(part 1 of 2)
# Autodesk Inventor assembly: Main
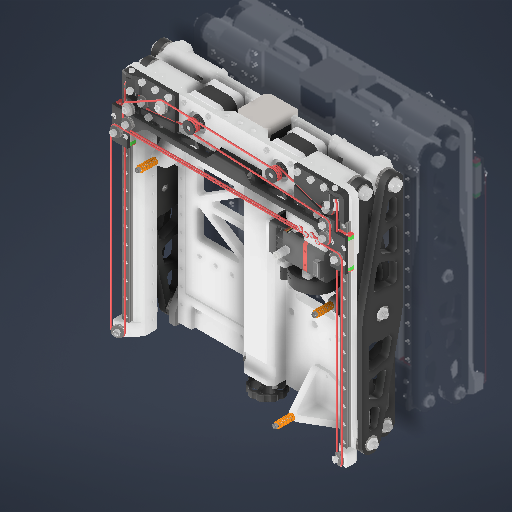
[picture p0: Inventor's stored thumbnail of the model, 512x512]
Saved by Autodesk Inventor 2026.2 (Build 302298000, 298)
## iProperties
Created: 2025-11-20
Part Number: Main
Document SubType Name: Assembly
Designer: gaoet
Author: gaoet
## Documents named in this file (83)
- C:\Users\gaoet\OneDrive\Desktop\Scissor 3D Printer\Main.iam
- C:\Users\gaoet\OneDrive\Desktop\Scissor 3D Printer\Zeee6S22Ah.ipt
- C:\Users\gaoet\Downloads\Positron V3.2.2\42SHD0034-20B\42SHD0034-20B.ipt
- C:\Users\gaoet\OneDrive\Desktop\Scissor 3D Printer\BoundingBox.ipt
- C:\Users\gaoet\OneDrive\Desktop\Scissor 3D Printer\BuildVolume.ipt
- C:\Users\gaoet\OneDrive\Desktop\Scissor 3D Printer\LaptopScaleModel.ipt
- C:\Users\gaoet\OneDrive\Desktop\Scissor 3D Printer\Raspberry PI Zero W\Raspberry PI Zero W.iam
- C:\Users\gaoet\OneDrive\Desktop\Scissor 3D Printer\BTT E3 SKR MINI V3.0\BTT E3 SKR MINI V3.0.iam
- C:\Users\gaoet\OneDrive\Desktop\Scissor 3D Printer\MGN9-H\MGN9-H\MGN9-H.ipt
- C:\Users\gaoet\OneDrive\Desktop\Scissor 3D Printer\ElectronicsBase.ipt
- C:\Users\gaoet\OneDrive\Desktop\Scissor 3D Printer\BottomSlideMount.ipt
- C:\Users\gaoet\OneDrive\Desktop\Scissor 3D Printer\Pololu Stepper with 300mm LeadScrew\Pololu Stepper with 300mm LeadScrew\Pololu Stepper with 300mm LeadScrew.ipt
- C:\Users\gaoet\OneDrive\Desktop\Scissor 3D Printer\nut TR8x8 v7\nut TR8x8 v7\nut TR8x8 v7.ipt
- C:\Users\gaoet\OneDrive\Desktop\Scissor 3D Printer\ZMotorMount.ipt
- C:\Users\gaoet\OneDrive\Desktop\Scissor 3D Printer\BottomSideMountRight.ipt
- C:\Users\gaoet\OneDrive\Desktop\Scissor 3D Printer\ZBridgePlate.ipt
- C:\Users\gaoet\OneDrive\Desktop\Scissor 3D Printer\ScissorArmV2.ipt
- C:\Users\gaoet\OneDrive\Desktop\Scissor 3D Printer\7804K117_Stainless Steel Ball Bearing\7804K117_Stainless Steel Ball Bearing\7804K117_Stainless Steel Ball Bearing.ipt
- C:\Users\gaoet\OneDrive\Desktop\Scissor 3D Printer\92981A207_Alloy Steel Shoulder Screws\92981A207_Alloy Steel Shoulder Screws\92981A207_Alloy Steel Shoulder Screws.ipt
- C:\Users\gaoet\OneDrive\Desktop\Scissor 3D Printer\ShoulderBoltMountV2.ipt
- C:\Users\gaoet\OneDrive\Desktop\Scissor 3D Printer\91415A210_Zinc-Plated Steel Hex Nut\91415A210_Zinc-Plated Steel Hex Nut\91415A210_Zinc-Plated Steel Hex Nut.ipt
- C:\Users\gaoet\OneDrive\Desktop\Scissor 3D Printer\CarriagePivotMount.ipt
- C:\Users\gaoet\OneDrive\Desktop\Scissor 3D Printer\91290A306_Black-Oxide Alloy Steel Socket Head Screw\91290A306_Black-Oxide Alloy Steel Socket Head Screw\91290A306_Black-Oxide Alloy Steel Socket Head Screw.ipt
- C:\Users\gaoet\OneDrive\Desktop\Scissor 3D Printer\PivotWasher.ipt
- C:\Users\gaoet\OneDrive\Desktop\Scissor 3D Printer\90591A255_Zinc-Plated Steel Hex Nut\90591A255_Zinc-Plated Steel Hex Nut\90591A255_Zinc-Plated Steel Hex Nut.ipt
- C:\Users\gaoet\OneDrive\Desktop\Scissor 3D Printer\ScissorArmV2Inner.ipt
- C:\Users\gaoet\OneDrive\Desktop\Scissor 3D Printer\6656K108_Steel Ball Bearing\6656K108_Steel Ball Bearing\6656K108_Steel Ball Bearing.ipt
- C:\Users\gaoet\OneDrive\Desktop\Scissor 3D Printer\91290A168_Black-Oxide Alloy Steel Socket Head Screw\91290A168_Black-Oxide Alloy Steel Socket Head Screw\91290A168_Black-Oxide Alloy Steel Socket Head Screw.ipt
- C:\Users\gaoet\OneDrive\Desktop\Scissor 3D Printer\ThrustBearing.iam
- C:\Users\gaoet\OneDrive\Desktop\Scissor 3D Printer\MGN9-C v2 v0\MGN9-C v2.iam
- C:\Users\gaoet\OneDrive\Desktop\Scissor 3D Printer\UpperCarriagePivotMount.ipt
- C:\Users\gaoet\OneDrive\Desktop\Scissor 3D Printer\MGN9-H\MGN9-H\MGN9-H_MIR.ipt
- C:\Users\gaoet\OneDrive\Desktop\Scissor 3D Printer\91415A210_Zinc-Plated Steel Hex Nut\91415A210_Zinc-Plated Steel Hex Nut\91415A210_Zinc-Plated Steel Hex Nut_MIR.ipt
- C:\Users\gaoet\OneDrive\Desktop\Scissor 3D Printer\7804K117_Stainless Steel Ball Bearing\7804K117_Stainless Steel Ball Bearing\7804K117_Stainless Steel Ball Bearing_MIR.ipt
- C:\Users\gaoet\OneDrive\Desktop\Scissor 3D Printer\ScissorArmV2_MIR.ipt
- C:\Users\gaoet\OneDrive\Desktop\Scissor 3D Printer\92981A207_Alloy Steel Shoulder Screws\92981A207_Alloy Steel Shoulder Screws\92981A207_Alloy Steel Shoulder Screws_MIR.ipt
- C:\Users\gaoet\OneDrive\Desktop\Scissor 3D Printer\CarriagePivotMount_MIR.ipt
- C:\Users\gaoet\OneDrive\Desktop\Scissor 3D Printer\91290A306_Black-Oxide Alloy Steel Socket Head Screw\91290A306_Black-Oxide Alloy Steel Socket Head Screw\91290A306_Black-Oxide Alloy Steel Socket Head Screw_MIR.ipt
- C:\Users\gaoet\OneDrive\Desktop\Scissor 3D Printer\PivotWasher_MIR.ipt
- C:\Users\gaoet\OneDrive\Desktop\Scissor 3D Printer\90591A255_Zinc-Plated Steel Hex Nut\90591A255_Zinc-Plated Steel Hex Nut\90591A255_Zinc-Plated Steel Hex Nut_MIR.ipt
- C:\Users\gaoet\OneDrive\Desktop\Scissor 3D Printer\ScissorArmV2Inner_MIR.ipt
- C:\Users\gaoet\OneDrive\Desktop\Scissor 3D Printer\6656K108_Steel Ball Bearing\6656K108_Steel Ball Bearing\6656K108_Steel Ball Bearing_MIR.ipt
- C:\Users\gaoet\OneDrive\Desktop\Scissor 3D Printer\91290A168_Black-Oxide Alloy Steel Socket Head Screw\91290A168_Black-Oxide Alloy Steel Socket Head Screw\91290A168_Black-Oxide Alloy Steel Socket Head Screw_MIR.ipt
- C:\Users\gaoet\OneDrive\Desktop\Scissor 3D Printer\ThrustBearing_MIR.iam
- C:\Users\gaoet\OneDrive\Desktop\Scissor 3D Printer\MGN9-C v2 v0\MGN9-C v2_MIR.iam
- C:\Users\gaoet\OneDrive\Desktop\Scissor 3D Printer\UpperCarriagePivotMount_MIR.ipt
- C:\Users\gaoet\OneDrive\Desktop\Scissor 3D Printer\91290A110_Black-Oxide Alloy Steel Socket Head Screw\91290A110_Black-Oxide Alloy Steel Socket Head Screw\91290A110_Black-Oxide Alloy Steel Socket Head Screw_MIR.ipt
- C:\Users\gaoet\OneDrive\Desktop\Scissor 3D Printer\GantryRailMount_MIR.ipt
- C:\Users\gaoet\OneDrive\Desktop\Scissor 3D Printer\Extruder.iam
- C:\Users\gaoet\OneDrive\Desktop\Scissor 3D Printer\MGNRail250mm.ipt
- C:\Users\gaoet\OneDrive\Desktop\Scissor 3D Printer\XGantryMount.ipt
- C:\Users\gaoet\OneDrive\Desktop\Scissor 3D Printer\BearingU604.ipt
- C:\Users\gaoet\OneDrive\Desktop\Scissor 3D Printer\90729A168_Passivated 316 Stainless Steel Hex-Drive Flat Head Screw\90729A168_Passivated 316 Stainless Steel Hex-Drive Flat Head Screw\90729A168_Passivated 316 .ipt
- C:\Users\gaoet\OneDrive\Desktop\Scissor 3D Printer\ElevatorPlate.ipt
- C:\Users\gaoet\OneDrive\Desktop\Scissor 3D Printer\ElevatorPlate_MIR.ipt
- C:\Users\gaoet\OneDrive\Desktop\Scissor 3D Printer\XGantryMount_MIR.ipt
- C:\Users\gaoet\OneDrive\Desktop\Scissor 3D Printer\ElevatorShoulderBoltMount.ipt
- C:\Users\gaoet\OneDrive\Desktop\Scissor 3D Printer\ElevatorShoulderBoltMount_MIR.ipt
- C:\Users\gaoet\OneDrive\Desktop\Scissor 3D Printer\Pulley.ipt
- C:\Users\gaoet\OneDrive\Desktop\Scissor 3D Printer\Tensioner.ipt
- C:\Users\gaoet\OneDrive\Desktop\Scissor 3D Printer\PSU.ipt
- C:\Users\gaoet\OneDrive\Desktop\Scissor 3D Printer\LeadScrewArch.ipt
- C:\Users\gaoet\OneDrive\Desktop\Scissor 3D Printer\FrontPanel.ipt
- C:\Users\gaoet\OneDrive\Desktop\Scissor 3D Printer\knob.ipt
- C:\Users\gaoet\OneDrive\Desktop\Scissor 3D Printer\BTT Mini 12864 V1.0\BTT Mini 12864 V1.0\BTT Mini 12864 V1.0.ipt
- C:\Users\gaoet\OneDrive\Desktop\Scissor 3D Printer\BottomSlideMountExtension.ipt
- C:\Users\gaoet\OneDrive\Desktop\Scissor 3D Printer\BottomSlideMountExtension_MIR.ipt
- C:\Users\gaoet\OneDrive\Desktop\Scissor 3D Printer\RightTruss.ipt
- C:\Users\gaoet\OneDrive\Desktop\Scissor 3D Printer\LeftTruss.ipt
- C:\Users\gaoet\OneDrive\Desktop\Scissor 3D Printer\RoutingPlateV2.ipt
- C:\Users\gaoet\OneDrive\Desktop\Scissor 3D Printer\RoutingPlateV2Right.ipt
- C:\Users\gaoet\OneDrive\Desktop\Scissor 3D Printer\ShoulderBoltMountV2_MIR.ipt
- C:\Users\gaoet\OneDrive\Desktop\Scissor 3D Printer\92095A181_NO THREADS_18-8 Stainless Steel Button Head Hex-Drive Screw\92095A181_NO THREADS_18-8 Stainless Steel Button Head Hex-Drive Screw\92095A181_NO THREAD.ipt
- C:\Users\gaoet\OneDrive\Desktop\Scissor 3D Printer\MockCable.ipt
- C:\Users\gaoet\OneDrive\Desktop\Scissor 3D Printer\MockCable2.ipt
- C:\Users\gaoet\OneDrive\Desktop\Scissor 3D Printer\Banana\Banana\Banana.ipt
- C:\Users\gaoet\OneDrive\Desktop\Scissor 3D Printer\GantryRailMount.ipt
- C:\Users\gaoet\OneDrive\Desktop\Scissor 3D Printer\cardboard spool v1\cardboard spool v1\cardboard spool v1.ipt
- C:\Users\gaoet\OneDrive\Desktop\Scissor 3D Printer\LeftLevelBlock.ipt
- C:\Users\gaoet\OneDrive\Desktop\Scissor 3D Printer\RightLevelBlock.ipt
- C:\Users\gaoet\OneDrive\Desktop\Scissor 3D Printer\FrontLevelBlock.ipt
- C:\Users\gaoet\OneDrive\Desktop\Scissor 3D Printer\Spring8x20mm.ipt
- C:\Users\gaoet\OneDrive\Desktop\Polar Plotter\91290A123_Alloy Steel Socket Head Screw\91290A123_Alloy Steel Socket Head Screw.ipt
## Components (336 placed, 82 different names)
1. Zeee6S22Ah:1 — Mate:155, Mate:167
2. 42SHD0034-20B:1 — Mate:132, Flush:39, Mate:143, Mate:148, Flush:46
3. BoundingBox:1 — Mate:41, Flush:14, Mate:42, Angle:2, Mate:149, Flush:47
4. BuildVolume:1
5. LaptopScaleModel:1
6. Raspberry PI Zero W:1 [sub-assembly] — Insert:233, Mate:166, Insert:264, Insert:265
7. BTT E3 SKR MINI V3.0:1 [sub-assembly] — Insert:234, Mate:169
8. MGN9-H:2 — Insert:39, Mate:61, Mate:185
9. MGN9-H:3 — Mate:111, Flush:33, Insert:310
10. MGN9-H:6 — Mate:112, Flush:30, Insert:123, Mate:116
11. ElectronicsBase:1 — Mate:149, Flush:47, Mate:156, Flush:49, Insert:203, Insert:206, Insert:210, Insert:214, Insert:215
12. BottomSlideMount:1 — Mate:13, Mate:20, Insert:10, Insert:11, Mate:139, Mate:140, Flush:43, Insert:207, Insert:208, Insert:213, Mate:167, Mate:170, Mate:171, Flush:50, Insert:261, Insert:328, Flush:53
13. Pololu Stepper with 300mm LeadScrew:1 — Mate:11, Insert:2, Insert:3, Mate:41, Mate:42, Mate:152
14. nut TR8x8 v7:1 — Mate:11, Angle:1
15. ZMotorMount:1 — Insert:2, Insert:3, Mate:13, Mate:20, Mate:22, Insert:10, Insert:11, Mate:23, Mate:24, Angle:1, Mate:72, Mate:82, Mate:154, Insert:266, Insert:267, Insert:268, Insert:269, Insert:270, Insert:271, Insert:272, Insert:303
16. BottomSideMountRight:1 — Mate:22, Mate:23, Mate:24, Flush:14, Mate:52, Mate:53, Mate:54, Angle:8, Mate:138, Mate:141, Mate:153, Mate:168, Mate:169, Mate:172, Insert:283, Flush:52, Insert:329, Flush:54
17. ZBridgePlate:1 — Insert:40, Mate:72, Mate:82, Insert:137, Insert:300, Insert:301, Insert:302
18. 91415A210_Zinc-Plated Steel Hex Nut:1 — Mate:56, Mate:57
19. 7804K117_Stainless Steel Ball Bearing:2 — Mate:70, Insert:52, Insert:325
20. ScissorArmV2:3 — Insert:35, Angle:2, Mate:73, Insert:63, Insert:64, Insert:71, Insert:74, Insert:78, Angle:4
21. 7804K117_Stainless Steel Ball Bearing:3 — Insert:35, Insert:37
22. 92981A207_Alloy Steel Shoulder Screws:3 — Insert:37, Mate:56
23. ShoulderBoltMountV2:1 — Mate:52, Mate:53, Mate:54, Mate:57, Insert:70, Insert:273, Insert:274, Insert:275, Insert:276, Insert:277, Insert:290, Insert:291
24. CarriagePivotMount:1 — Insert:39, Mate:61, Insert:40, Insert:53, Insert:72
25. 91290A306_Black-Oxide Alloy Steel Socket Head Screw:1 — Mate:70, Insert:51
26. PivotWasher:1 — Insert:51, Insert:52
27. 90591A255_Zinc-Plated Steel Hex Nut:1 — Insert:53
28. ScissorArmV2Inner:1 — Mate:73, Insert:68, Mate:74, Insert:73, Angle:4, Insert:316, Insert:325, Insert:326
29. 7804K117_Stainless Steel Ball Bearing:6 — Insert:63, Insert:66
30. 6656K108_Steel Ball Bearing:1 — Insert:64, Insert:65
31. 6656K108_Steel Ball Bearing:2 — Insert:65
32. PivotWasher:3 — Insert:66, Insert:67
33. 91290A168_Black-Oxide Alloy Steel Socket Head Screw:2 — Insert:67
34. 90591A255_Zinc-Plated Steel Hex Nut:2 — Insert:68, Mate:74
35. ThrustBearing:1 [sub-assembly] — Insert:70, Insert:71
36. ThrustBearing:2 [sub-assembly] — Insert:72, Insert:73
37. MGN9-C v2:1 [sub-assembly] — Mate:80, Insert:308, Flush:51
38. 7804K117_Stainless Steel Ball Bearing:7 — Insert:74, Insert:76
39. PivotWasher:4 — Insert:76, Insert:88
40. ThrustBearing:3 [sub-assembly] — Insert:78, Mate:77, Mate:78
41. UpperCarriagePivotMount:1 — Mate:77, Mate:78, Mate:80, Insert:89, Mate:89, Insert:292, Insert:293, Insert:294, Insert:295, Insert:308
42. 91290A306_Black-Oxide Alloy Steel Socket Head Screw:3 — Insert:88
43. 90591A255_Zinc-Plated Steel Hex Nut:3 — Insert:89, Mate:89
44. MGN9-H_MIR:1 — Mate:94, Insert:93
45. 91415A210_Zinc-Plated Steel Hex Nut_MIR:1 — Mate:93
46. 7804K117_Stainless Steel Ball Bearing_MIR:1 — Mate:95, Insert:94, Insert:324
47. ScissorArmV2_MIR:1 — Insert:90, Angle:6, Mate:96, Insert:98, Insert:99, Insert:104, Insert:107, Insert:109
48. 7804K117_Stainless Steel Ball Bearing_MIR:2 — Insert:90, Insert:91
49. 92981A207_Alloy Steel Shoulder Screws_MIR:1 — Mate:93, Insert:91
50. CarriagePivotMount_MIR:1 — Mate:94, Insert:93, Insert:96, Insert:106, Insert:137
51. 91290A306_Black-Oxide Alloy Steel Socket Head Screw_MIR:1 — Mate:95, Insert:95
52. PivotWasher_MIR:1 — Insert:94, Insert:95
53. 90591A255_Zinc-Plated Steel Hex Nut_MIR:1 — Insert:96
54. ScissorArmV2Inner_MIR:1 — Angle:6, Mate:96, Mate:97, Insert:103, Insert:105, Insert:317, Insert:324, Insert:327, Mate:186
55. 7804K117_Stainless Steel Ball Bearing_MIR:3 — Insert:98, Insert:101
56. 6656K108_Steel Ball Bearing_MIR:1 — Insert:99, Insert:100
57. 6656K108_Steel Ball Bearing_MIR:2 — Insert:100, Mate:186
58. PivotWasher_MIR:2 — Insert:101, Insert:102
59. 91290A168_Black-Oxide Alloy Steel Socket Head Screw_MIR:1 — Insert:102
60. 90591A255_Zinc-Plated Steel Hex Nut_MIR:2 — Mate:97, Insert:103
61. ThrustBearing_MIR:1 [sub-assembly] — Insert:104, Insert:241
62. ThrustBearing_MIR:2 [sub-assembly] — Insert:105, Insert:106
63. MGN9-C v2_MIR:1 [sub-assembly] — Mate:99, Mate:122, Flush:35, Insert:307
64. 7804K117_Stainless Steel Ball Bearing_MIR:4 — Insert:107, Insert:108
65. PivotWasher_MIR:3 — Insert:108, Insert:116
66. ThrustBearing_MIR:3 [sub-assembly] — Insert:109, Mate:100, Mate:101
67. UpperCarriagePivotMount_MIR:1 — Mate:99, Mate:100, Mate:101, Mate:106, Insert:117, Insert:296, Insert:297, Insert:298, Insert:299, Insert:307
68. 91290A306_Black-Oxide Alloy Steel Socket Head Screw_MIR:2 — Insert:116
69. 90591A255_Zinc-Plated Steel Hex Nut_MIR:3 — Mate:106, Insert:117
70. Extruder:1 [sub-assembly] — Insert:310, Insert:311, Insert:312, Insert:313, Insert:314
71. MGNRail250mm:3 — Angle:8, Mate:111, Insert:124, Flush:33, Mate:117, Insert:260
72. MGNRail250mm:4 — Mate:112, Flush:30, Insert:152, Mate:128, Insert:319, Insert:320
73. XGantryMount:1 — Insert:123, Mate:116, Insert:124, Mate:117, Insert:138, Insert:139, Insert:140, Insert:141, Mate:126, Insert:142, Insert:145, Mate:131, Flush:42, Insert:183, Insert:184, Mate:174, Angle:12
74. GantryRailMount_MIR:1 — Insert:132, Insert:133, Insert:134, Insert:135, Insert:153
75. MGNRail250mm:6 — Mate:122, Flush:35, Insert:132, Insert:133, Insert:287
76. MGN9-H:7 — Insert:154, Mate:135
77. MGNRail250mm:7 — Insert:134, Insert:135, Insert:247, Mate:188
78. BearingU604:1 — Insert:147, Insert:321
79. BearingU604:2 — Insert:145, Insert:146
80. BearingU604:3 — Mate:126, Insert:142, Insert:143
81. BearingU604:4 — Insert:156, Insert:158, Mate:178
82. BearingU604:5 — Insert:155, Insert:159
83. BearingU604:6 — Insert:153, Insert:157, Mate:179
84. 90729A168_Passivated 316 :1 — Insert:140
85. 90729A168_Passivated 316 :2 — Insert:141
86. 90729A168_Passivated 316 :3 — Insert:139
87. 90729A168_Passivated 316 :4 — Insert:138
88. 91290A306_Black-Oxide Alloy Steel Socket Head Screw:4 — Insert:143, Mate:175
89. 91290A306_Black-Oxide Alloy Steel Socket Head Screw:5 — Insert:146
90. 91290A306_Black-Oxide Alloy Steel Socket Head Screw:6 — Insert:147
91. 90729A168_Passivated 316 :5 — Insert:312
92. 90729A168_Passivated 316 :6 — Insert:313
93. 90729A168_Passivated 316 :7 — Mate:173, Insert:314
94. 90729A168_Passivated 316 :8 — Insert:311
95. ElevatorPlate:1 — Insert:152, Mate:128, Mate:129, Angle:10, Mate:131, Flush:40, Flush:41, Mate:136, Mate:147, Insert:216, Insert:217, Insert:258, Mate:180, Insert:322, Insert:323
96. 42SHD0034-20B:4 — Mate:129, Angle:10, Mate:142, Flush:45, Mate:147
97. ElevatorPlate_MIR:1 — Mate:132, Flush:39, Flush:40, Flush:41, Insert:182, Mate:148, Insert:223, Insert:259, Mate:180, Mate:184, Mate:188
98. XGantryMount_MIR:1 — Insert:154, Mate:135, Flush:42, Insert:155, Insert:156, Insert:160, Insert:161, Insert:162, Insert:163
99. 91290A306_Black-Oxide Alloy Steel Socket Head Screw:7 — Insert:157
100. 91290A306_Black-Oxide Alloy Steel Socket Head Screw:8 — Insert:158
101. 91290A306_Black-Oxide Alloy Steel Socket Head Screw:9 — Insert:159
102. 90729A168_Passivated 316 :9 — Insert:163
103. 90729A168_Passivated 316 :10 — Insert:162
104. 90729A168_Passivated 316 :11 — Insert:161
105. 90729A168_Passivated 316 :12 — Insert:160
106. 92981A207_Alloy Steel Shoulder Screws:4 — Insert:165
107. ThrustBearing:4 [sub-assembly] — Insert:315, Insert:316
108. 7804K117_Stainless Steel Ball Bearing:8 — Insert:165, Insert:326
109. ElevatorShoulderBoltMount:1 — Mate:136, Insert:315, Insert:318
110. 91415A210_Zinc-Plated Steel Hex Nut:3 — Insert:318
111. ElevatorShoulderBoltMount_MIR:1 — Insert:182, Mate:163, Mate:181, Mate:184
112. 92981A207_Alloy Steel Shoulder Screws:5 — Insert:176
113. ThrustBearing:5 [sub-assembly] — Insert:317, Mate:181
114. 7804K117_Stainless Steel Ball Bearing_MIR:5 — Insert:176, Insert:327
115. MGNRail250mm:8 — Mate:138, Mate:141, Mate:185
116. MGNRail250mm:9 — Mate:139, Mate:140, Flush:43, Insert:285
117. BearingU604:10 — Insert:218, Insert:219
118. BearingU604:12 — Insert:187
119. 91290A306_Black-Oxide Alloy Steel Socket Head Screw:20 — Insert:184
120. 91290A306_Black-Oxide Alloy Steel Socket Head Screw:21 — Insert:183
121. Pulley:1 — Mate:142, Flush:45
122. Pulley:2 — Mate:143, Flush:46
123. BearingU604:17 — Insert:229, Insert:231
124. Tensioner:1 — Insert:187, Mate:159, Insert:220, Mate:176, Mate:182
125. PSU:1
126. LeadScrewArch:1 — Mate:152, Mate:153, Mate:154, Insert:194, Mate:155, Insert:263, Insert:306
127. 7804K117_Stainless Steel Ball Bearing:9 — Insert:194
128. knob:1 — Insert:198
129. FrontPanel:2 — Mate:156, Flush:49, Insert:197, Angle:11, Insert:199, Insert:200, Insert:201, Insert:202, Insert:243, Insert:244, Insert:245, Insert:246
130. 7804K117_Stainless Steel Ball Bearing:10 — Insert:197, Insert:198
131. 90729A168_Passivated 316 :13 — Insert:201
132. 90729A168_Passivated 316 :14 — Insert:202
133. BTT Mini 12864 V1.0:1 — Angle:11, Insert:199, Insert:200
134. 90729A168_Passivated 316 :15 — Insert:203
135. 90729A168_Passivated 316 :16 — Insert:206
136. 90729A168_Passivated 316 :17 — Insert:210
137. BottomSlideMountExtension:1 — Insert:207, Insert:208, Insert:212, Insert:233, Mate:166
138. BottomSlideMountExtension_MIR:1 — Insert:211, Insert:234, Mate:168, Mate:172, Insert:284, Insert:330, Mate:187
139. RightTruss:1 — Insert:211, Flush:52
140. LeftTruss:1 — Insert:212, Insert:213
141. 90729A168_Passivated 316 :19 — Insert:214
142. 90729A168_Passivated 316 :20 — Insert:215
143. RoutingPlateV2:1 — Insert:216, Insert:217, Mate:159, Insert:218, Insert:221, Insert:248, Insert:249, Insert:250, Insert:251, Insert:257, Mate:176, Mate:182
144. 91290A306_Black-Oxide Alloy Steel Socket Head Screw:22 — Insert:219
145. 91290A306_Black-Oxide Alloy Steel Socket Head Screw:23 — Insert:220
146. BearingU604:18 — Insert:221, Insert:222
147. 91290A306_Black-Oxide Alloy Steel Socket Head Screw:24 — Insert:222
148. RoutingPlateV2Right:1 — Insert:223, Mate:163, Insert:225, Mate:164, Insert:228, Insert:229, Insert:252, Insert:253, Insert:254, Insert:255, Insert:256, Mate:177, Mate:183
149. BearingU604:19 — Insert:225, Insert:232
150. BearingU604:21
151. Tensioner:2 — Mate:164, Mate:177, Mate:183
152. 91290A306_Black-Oxide Alloy Steel Socket Head Screw:25
153. BearingU604:22 — Insert:228, Insert:230
154. 91290A306_Black-Oxide Alloy Steel Socket Head Screw:26 — Insert:230
155. 91290A306_Black-Oxide Alloy Steel Socket Head Screw:27 — Insert:231
156. 91290A306_Black-Oxide Alloy Steel Socket Head Screw:28 — Insert:232
157. ShoulderBoltMountV2_MIR:1 — Insert:241, Mate:170, Mate:171, Flush:50, Insert:278, Insert:279, Insert:280, Insert:281, Insert:282, Insert:288, Insert:289
158. 90729A168_Passivated 316 :28 — Insert:243
159. 90729A168_Passivated 316 :29 — Insert:244
160. 90729A168_Passivated 316 :30 — Insert:245
161. 90729A168_Passivated 316 :31 — Insert:246
162. 91290A306_Black-Oxide Alloy Steel Socket Head Screw:29 — Insert:249
163. 91290A306_Black-Oxide Alloy Steel Socket Head Screw:30 — Insert:251
164. 91290A306_Black-Oxide Alloy Steel Socket Head Screw:31 — Insert:250
165. 91290A306_Black-Oxide Alloy Steel Socket Head Screw:32 — Insert:248
166. 91290A306_Black-Oxide Alloy Steel Socket Head Screw:33 — Insert:255
167. 91290A306_Black-Oxide Alloy Steel Socket Head Screw:34 — Insert:254
168. 91290A306_Black-Oxide Alloy Steel Socket Head Screw:35 — Insert:252
169. 91290A306_Black-Oxide Alloy Steel Socket Head Screw:36 — Insert:253
170. 91290A110_Black-Oxide Alloy Steel Socket Head Screw_MIR:31 — Insert:257
171. 91290A110_Black-Oxide Alloy Steel Socket Head Screw_MIR:32 — Insert:256
172. 91290A110_Black-Oxide Alloy Steel Socket Head Screw_MIR:60 — Insert:263
173. 91290A110_Black-Oxide Alloy Steel Socket Head Screw_MIR:61 — Insert:264
174. 91290A110_Black-Oxide Alloy Steel Socket Head Screw_MIR:62 — Insert:265
175. 91290A306_Black-Oxide Alloy Steel Socket Head Screw:38 — Insert:266
176. 91290A306_Black-Oxide Alloy Steel Socket Head Screw:39 — Insert:267
177. 91290A306_Black-Oxide Alloy Steel Socket Head Screw:40 — Insert:268
178. 91290A306_Black-Oxide Alloy Steel Socket Head Screw:41 — Insert:269
179. 91290A306_Black-Oxide Alloy Steel Socket Head Screw:42 — Insert:270
180. 91290A306_Black-Oxide Alloy Steel Socket Head Screw:43 — Insert:271
181. 91290A306_Black-Oxide Alloy Steel Socket Head Screw:44 — Insert:272
182. 91290A306_Black-Oxide Alloy Steel Socket Head Screw:46 — Insert:273
183. 91290A306_Black-Oxide Alloy Steel Socket Head Screw:47 — Insert:274
184. 91290A306_Black-Oxide Alloy Steel Socket Head Screw:48 — Insert:275
185. 91290A306_Black-Oxide Alloy Steel Socket Head Screw:49 — Insert:276
186. 91290A306_Black-Oxide Alloy Steel Socket Head Screw:50 — Insert:277
187. 91290A306_Black-Oxide Alloy Steel Socket Head Screw:51 — Insert:278
188. 91290A306_Black-Oxide Alloy Steel Socket Head Screw:52 — Insert:279
189. 91290A306_Black-Oxide Alloy Steel Socket Head Screw:53 — Insert:280
190. 91290A306_Black-Oxide Alloy Steel Socket Head Screw:54 — Insert:281
191. 91290A306_Black-Oxide Alloy Steel Socket Head Screw:55 — Insert:282
192. 91290A306_Black-Oxide Alloy Steel Socket Head Screw:60 — Insert:284
193. 91290A110_Black-Oxide Alloy Steel Socket Head Screw_MIR:115 — Insert:288
194. 91290A110_Black-Oxide Alloy Steel Socket Head Screw_MIR:116 — Insert:289
195. 91290A110_Black-Oxide Alloy Steel Socket Head Screw_MIR:117 — Insert:290
196. 91290A110_Black-Oxide Alloy Steel Socket Head Screw_MIR:118 — Insert:291
197. 92095A181_NO THREAD:1 — Insert:295
198. 92095A181_NO THREAD:2 — Insert:294
199. 92095A181_NO THREAD:3 — Insert:293
200. 92095A181_NO THREAD:4 — Insert:292
201. 92095A181_NO THREAD:5 — Insert:296
202. 92095A181_NO THREAD:6 — Insert:297
203. 92095A181_NO THREAD:7 — Insert:298
204. 92095A181_NO THREAD:8 — Insert:299
205. 91290A110_Black-Oxide Alloy Steel Socket Head Screw_MIR:123
206. 91290A110_Black-Oxide Alloy Steel Socket Head Screw_MIR:124
207. MockCable:1 — Mate:173, Mate:174, Angle:12, Mate:175
208. MockCable2:1 — Mate:178, Mate:179
209. Banana:1
210. GantryRailMount:1 — Insert:319, Insert:320, Insert:321
211. MGNRail250mm:10 — Insert:322, Insert:323, Flush:51
212. cardboard spool v1:1
213. LeftLevelBlock:1 — Insert:328, Flush:53, Insert:333
214. RightLevelBlock:1 — Insert:329, Flush:54, Insert:332
215. FrontLevelBlock:1 — Insert:330, Mate:187, Insert:331
216. Spring8x20mm:1 — Insert:331, Insert:334
217. Spring8x20mm:2 — Insert:333, Insert:335
218. Spring8x20mm:3 — Insert:332, Insert:336
219. Pololu Stepper with 300mm LeadScrew:2
220. 91290A123_Alloy Steel Socket Head Screw:1 — Insert:335
221. 91290A123_Alloy Steel Socket Head Screw:2 — Insert:336
222. 91290A123_Alloy Steel Socket Head Screw:3 — Insert:334
223. 91290A110_Black-Oxide Alloy Steel Socket Head Screw_MIR:5 — Insert:247
224. 91290A110_Black-Oxide Alloy Steel Socket Head Screw_MIR:18
225. 91290A110_Black-Oxide Alloy Steel Socket Head Screw_MIR:6
226. 91290A110_Black-Oxide Alloy Steel Socket Head Screw_MIR:19
227. 91290A110_Black-Oxide Alloy Steel Socket Head Screw_MIR:7
228. 91290A110_Black-Oxide Alloy Steel Socket Head Screw_MIR:20
229. 91290A110_Black-Oxide Alloy Steel Socket Head Screw_MIR:8
230. 91290A110_Black-Oxide Alloy Steel Socket Head Screw_MIR:21
231. 91290A110_Black-Oxide Alloy Steel Socket Head Screw_MIR:9
232. 91290A110_Black-Oxide Alloy Steel Socket Head Screw_MIR:22
233. 91290A110_Black-Oxide Alloy Steel Socket Head Screw_MIR:10
234. 91290A110_Black-Oxide Alloy Steel Socket Head Screw_MIR:23
235. 91290A110_Black-Oxide Alloy Steel Socket Head Screw_MIR:11
236. 91290A110_Black-Oxide Alloy Steel Socket Head Screw_MIR:24
237. 91290A110_Black-Oxide Alloy Steel Socket Head Screw_MIR:12
238. 91290A110_Black-Oxide Alloy Steel Socket Head Screw_MIR:25
239. 91290A110_Black-Oxide Alloy Steel Socket Head Screw_MIR:13
240. 91290A110_Black-Oxide Alloy Steel Socket Head Screw_MIR:26
241. 91290A110_Black-Oxide Alloy Steel Socket Head Screw_MIR:14
242. 91290A110_Black-Oxide Alloy Steel Socket Head Screw_MIR:27
243. 91290A110_Black-Oxide Alloy Steel Socket Head Screw_MIR:15
244. 91290A110_Black-Oxide Alloy Steel Socket Head Screw_MIR:28
245. 91290A110_Black-Oxide Alloy Steel Socket Head Screw_MIR:16
246. 91290A110_Black-Oxide Alloy Steel Socket Head Screw_MIR:29
247. 91290A110_Black-Oxide Alloy Steel Socket Head Screw_MIR:17
248. 91290A110_Black-Oxide Alloy Steel Socket Head Screw_MIR:30
249. 91290A110_Black-Oxide Alloy Steel Socket Head Screw_MIR:41 — Insert:260
250. 91290A110_Black-Oxide Alloy Steel Socket Head Screw_MIR:42
251. 91290A110_Black-Oxide Alloy Steel Socket Head Screw_MIR:43
252. 91290A110_Black-Oxide Alloy Steel Socket Head Screw_MIR:44
253. 91290A110_Black-Oxide Alloy Steel Socket Head Screw_MIR:45
254. 91290A110_Black-Oxide Alloy Steel Socket Head Screw_MIR:46
255. 91290A110_Black-Oxide Alloy Steel Socket Head Screw_MIR:47
256. 91290A110_Black-Oxide Alloy Steel Socket Head Screw_MIR:48
257. 91290A110_Black-Oxide Alloy Steel Socket Head Screw_MIR:49
258. 91290A110_Black-Oxide Alloy Steel Socket Head Screw_MIR:50
259. 91290A110_Black-Oxide Alloy Steel Socket Head Screw_MIR:51
260. 91290A110_Black-Oxide Alloy Steel Socket Head Screw_MIR:52
261. 91290A110_Black-Oxide Alloy Steel Socket Head Screw_MIR:53
262. 91290A110_Black-Oxide Alloy Steel Socket Head Screw_MIR:54 — Insert:261
263. 91290A110_Black-Oxide Alloy Steel Socket Head Screw_MIR:55
264. 91290A110_Black-Oxide Alloy Steel Socket Head Screw_MIR:56
265. 91290A306_Black-Oxide Alloy Steel Socket Head Screw:56 — Insert:283
266. 91290A306_Black-Oxide Alloy Steel Socket Head Screw:57
267. 91290A306_Black-Oxide Alloy Steel Socket Head Screw:58
268. 91290A306_Black-Oxide Alloy Steel Socket Head Screw:59
269. 91290A110_Black-Oxide Alloy Steel Socket Head Screw_MIR:63 — Insert:285
270. 91290A110_Black-Oxide Alloy Steel Socket Head Screw_MIR:64
271. 91290A110_Black-Oxide Alloy Steel Socket Head Screw_MIR:65
272. 91290A110_Black-Oxide Alloy Steel Socket Head Screw_MIR:66
273. 91290A110_Black-Oxide Alloy Steel Socket Head Screw_MIR:67
274. 91290A110_Black-Oxide Alloy Steel Socket Head Screw_MIR:68
275. 91290A110_Black-Oxide Alloy Steel Socket Head Screw_MIR:69
276. 91290A110_Black-Oxide Alloy Steel Socket Head Screw_MIR:70
277. 91290A110_Black-Oxide Alloy Steel Socket Head Screw_MIR:71
278. 91290A110_Black-Oxide Alloy Steel Socket Head Screw_MIR:72
279. 91290A110_Black-Oxide Alloy Steel Socket Head Screw_MIR:73
280. 91290A110_Black-Oxide Alloy Steel Socket Head Screw_MIR:74
281. 91290A110_Black-Oxide Alloy Steel Socket Head Screw_MIR:75
282. 91290A110_Black-Oxide Alloy Steel Socket Head Screw_MIR:76
283. 91290A110_Black-Oxide Alloy Steel Socket Head Screw_MIR:77
284. 91290A110_Black-Oxide Alloy Steel Socket Head Screw_MIR:78
285. 91290A110_Black-Oxide Alloy Steel Socket Head Screw_MIR:79
286. 91290A110_Black-Oxide Alloy Steel Socket Head Screw_MIR:80
287. 91290A110_Black-Oxide Alloy Steel Socket Head Screw_MIR:81
288. 91290A110_Black-Oxide Alloy Steel Socket Head Screw_MIR:82
289. 91290A110_Black-Oxide Alloy Steel Socket Head Screw_MIR:83
290. 91290A110_Black-Oxide Alloy Steel Socket Head Screw_MIR:84
291. 91290A110_Black-Oxide Alloy Steel Socket Head Screw_MIR:85
292. 91290A110_Black-Oxide Alloy Steel Socket Head Screw_MIR:86
293. 91290A110_Black-Oxide Alloy Steel Socket Head Screw_MIR:87
294. 91290A110_Black-Oxide Alloy Steel Socket Head Screw_MIR:88
295. 91290A110_Black-Oxide Alloy Steel Socket Head Screw_MIR:102 — Insert:287
296. 91290A110_Black-Oxide Alloy Steel Socket Head Screw_MIR:103
297. 91290A110_Black-Oxide Alloy Steel Socket Head Screw_MIR:104
298. 91290A110_Black-Oxide Alloy Steel Socket Head Screw_MIR:105
299. 91290A110_Black-Oxide Alloy Steel Socket Head Screw_MIR:106
300. 91290A110_Black-Oxide Alloy Steel Socket Head Screw_MIR:107
301. 91290A110_Black-Oxide Alloy Steel Socket Head Screw_MIR:108
302. 91290A110_Black-Oxide Alloy Steel Socket Head Screw_MIR:109
303. 91290A110_Black-Oxide Alloy Steel Socket Head Screw_MIR:110
304. 91290A110_Black-Oxide Alloy Steel Socket Head Screw_MIR:111
305. 91290A110_Black-Oxide Alloy Steel Socket Head Screw_MIR:112
306. 91290A110_Black-Oxide Alloy Steel Socket Head Screw_MIR:113
307. 91290A110_Black-Oxide Alloy Steel Socket Head Screw_MIR:114
308. 92095A181_NO THREAD:9 — Insert:300
309. 92095A181_NO THREAD:12
310. 92095A181_NO THREAD:13
311. 92095A181_NO THREAD:14
312. 92095A181_NO THREAD:10 — Insert:302
313. 92095A181_NO THREAD:15
314. 92095A181_NO THREAD:16
315. 92095A181_NO THREAD:17
316. 92095A181_NO THREAD:11 — Insert:301
317. 92095A181_NO THREAD:18
318. 92095A181_NO THREAD:19
319. 92095A181_NO THREAD:20
320. 91290A110_Black-Oxide Alloy Steel Socket Head Screw_MIR:119 — Insert:303
321. 91290A110_Black-Oxide Alloy Steel Socket Head Screw_MIR:120
322. 91290A110_Black-Oxide Alloy Steel Socket Head Screw_MIR:121
323. 91290A110_Black-Oxide Alloy Steel Socket Head Screw_MIR:122
324. 91290A110_Black-Oxide Alloy Steel Socket Head Screw_MIR:125 — Insert:306
325. 91290A110_Black-Oxide Alloy Steel Socket Head Screw_MIR:126
326. 91290A110_Black-Oxide Alloy Steel Socket Head Screw_MIR:127
327. 91290A110_Black-Oxide Alloy Steel Socket Head Screw_MIR:128
328. 91290A110_Black-Oxide Alloy Steel Socket Head Screw_MIR:129
329. 91290A110_Black-Oxide Alloy Steel Socket Head Screw_MIR:33 — Insert:258
330. 91290A110_Black-Oxide Alloy Steel Socket Head Screw_MIR:130
331. 91290A110_Black-Oxide Alloy Steel Socket Head Screw_MIR:131
332. 91290A110_Black-Oxide Alloy Steel Socket Head Screw_MIR:132
333. 91290A110_Black-Oxide Alloy Steel Socket Head Screw_MIR:37 — Insert:259
334. 91290A110_Black-Oxide Alloy Steel Socket Head Screw_MIR:133
335. 91290A110_Black-Oxide Alloy Steel Socket Head Screw_MIR:134
336. 91290A110_Black-Oxide Alloy Steel Socket Head Screw_MIR:135
## Component patterns: (26 elements, first: 91290A110_Black-Oxide Alloy Steel Socket Head Screw_MIR:5), (13 elements, first: 91290A110_Black-Oxide Alloy Steel Socket Head Screw_MIR:41), (3 elements, first: 91290A110_Black-Oxide Alloy Steel Socket Head Screw_MIR:54), (4 elements, first: 91290A306_Black-Oxide Alloy Steel Socket Head Screw:56), (26 elements, first: 91290A110_Black-Oxide Alloy Steel Socket Head Screw_MIR:63), (13 elements, first: 91290A110_Black-Oxide Alloy Steel Socket Head Screw_MIR:102), (4 elements, first: 92095A181_NO THREAD:9), (4 elements, first: 92095A181_NO THREAD:10), (4 elements, first: 92095A181_NO THREAD:11), (4 elements, first: 91290A110_Black-Oxide Alloy Steel Socket Head Screw_MIR:119), (5 elements, first: 91290A110_Black-Oxide Alloy Steel Socket Head Screw_MIR:125), (4 elements, first: 91290A110_Black-Oxide Alloy Steel Socket Head Screw_MIR:33), (4 elements, first: 91290A110_Black-Oxide Alloy Steel Socket Head Screw_MIR:37)
## Relationships (317: Insert 205, Mate 85, Flush 19, Angle 8)
- Mate:11: Pololu Stepper with 300mm LeadScrew:1 ↔ nut TR8x8 v7:1
- Insert:2: Pololu Stepper with 300mm LeadScrew:1 ↔ ZMotorMount:1
- Insert:3: Pololu Stepper with 300mm LeadScrew:1 ↔ ZMotorMount:1
- Mate:13: BottomSlideMount:1 ↔ ZMotorMount:1
- Mate:20: BottomSlideMount:1 ↔ ZMotorMount:1
- Mate:22: ZMotorMount:1 ↔ BottomSideMountRight:1
- Insert:10: BottomSlideMount:1 ↔ ZMotorMount:1
- Insert:11: BottomSlideMount:1 ↔ ZMotorMount:1
- Mate:23: ZMotorMount:1 ↔ BottomSideMountRight:1
- Mate:24: ZMotorMount:1 ↔ BottomSideMountRight:1
- Angle:1 (0 deg): nut TR8x8 v7:1 ↔ ZMotorMount:1
- Mate:41: BoundingBox:1 ↔ Pololu Stepper with 300mm LeadScrew:1
- Flush:14 (14 mm): BoundingBox:1 ↔ BottomSideMountRight:1
- Mate:42: BoundingBox:1 ↔ Pololu Stepper with 300mm LeadScrew:1
- Insert:35: ScissorArmV2:3 ↔ 7804K117_Stainless Steel Ball Bearing:3
- Insert:37: 7804K117_Stainless Steel Ball Bearing:3 ↔ 92981A207_Alloy Steel Shoulder Screws:3
- Mate:52: BottomSideMountRight:1 ↔ ShoulderBoltMountV2:1
- Mate:53: BottomSideMountRight:1 ↔ ShoulderBoltMountV2:1
- Mate:54: BottomSideMountRight:1 ↔ ShoulderBoltMountV2:1
- Mate:56: 91415A210_Zinc-Plated Steel Hex Nut:1 ↔ 92981A207_Alloy Steel Shoulder Screws:3
- Mate:57: 91415A210_Zinc-Plated Steel Hex Nut:1 ↔ ShoulderBoltMountV2:1
- Angle:2 (186 deg): BoundingBox:1 ↔ ScissorArmV2:3
- Insert:39: MGN9-H:2 ↔ CarriagePivotMount:1
- Mate:61: MGN9-H:2 ↔ CarriagePivotMount:1
- Insert:40: ZBridgePlate:1 ↔ CarriagePivotMount:1
- Mate:70: 7804K117_Stainless Steel Ball Bearing:2 ↔ 91290A306_Black-Oxide Alloy Steel Socket Head Screw:1
- Insert:51: 91290A306_Black-Oxide Alloy Steel Socket Head Screw:1 ↔ PivotWasher:1
- Insert:52: 7804K117_Stainless Steel Ball Bearing:2 ↔ PivotWasher:1
- Insert:53: CarriagePivotMount:1 ↔ 90591A255_Zinc-Plated Steel Hex Nut:1
- Mate:72: ZMotorMount:1 ↔ ZBridgePlate:1
- Mate:73: ScissorArmV2:3 ↔ ScissorArmV2Inner:1
- Insert:63: ScissorArmV2:3 ↔ 7804K117_Stainless Steel Ball Bearing:6
- Insert:64: ScissorArmV2:3 ↔ 6656K108_Steel Ball Bearing:1
- Insert:65: 6656K108_Steel Ball Bearing:1 ↔ 6656K108_Steel Ball Bearing:2
- Insert:66: 7804K117_Stainless Steel Ball Bearing:6 ↔ PivotWasher:3
- Insert:67: PivotWasher:3 ↔ 91290A168_Black-Oxide Alloy Steel Socket Head Screw:2
- Insert:68: ScissorArmV2Inner:1 ↔ 90591A255_Zinc-Plated Steel Hex Nut:2
- Mate:74: ScissorArmV2Inner:1 ↔ 90591A255_Zinc-Plated Steel Hex Nut:2
- Insert:70: ShoulderBoltMountV2:1 ↔ ThrustBearing:1
- Insert:71: ScissorArmV2:3 ↔ ThrustBearing:1
- Insert:72: CarriagePivotMount:1 ↔ ThrustBearing:2
- Insert:73: ScissorArmV2Inner:1 ↔ ThrustBearing:2
- Insert:74: ScissorArmV2:3 ↔ 7804K117_Stainless Steel Ball Bearing:7
- Insert:76: 7804K117_Stainless Steel Ball Bearing:7 ↔ PivotWasher:4
- Insert:78: ScissorArmV2:3 ↔ ThrustBearing:3
- Mate:77: ThrustBearing:3 ↔ UpperCarriagePivotMount:1
- Mate:78: ThrustBearing:3 ↔ UpperCarriagePivotMount:1
- Angle:4 (0 deg): ScissorArmV2:3 ↔ ScissorArmV2Inner:1
- Mate:80: MGN9-C v2:1 ↔ UpperCarriagePivotMount:1
- Mate:82 (178.4935 mm): ZMotorMount:1 ↔ ZBridgePlate:1
- Insert:88: PivotWasher:4 ↔ 91290A306_Black-Oxide Alloy Steel Socket Head Screw:3
- Insert:89: UpperCarriagePivotMount:1 ↔ 90591A255_Zinc-Plated Steel Hex Nut:3
- Mate:89: UpperCarriagePivotMount:1 ↔ 90591A255_Zinc-Plated Steel Hex Nut:3
- Insert:90: ScissorArmV2_MIR:1 ↔ 7804K117_Stainless Steel Ball Bearing_MIR:2
- Mate:93: 91415A210_Zinc-Plated Steel Hex Nut_MIR:1 ↔ 92981A207_Alloy Steel Shoulder Screws_MIR:1
- Insert:91: 7804K117_Stainless Steel Ball Bearing_MIR:2 ↔ 92981A207_Alloy Steel Shoulder Screws_MIR:1
- Mate:94: MGN9-H_MIR:1 ↔ CarriagePivotMount_MIR:1
- Insert:93: MGN9-H_MIR:1 ↔ CarriagePivotMount_MIR:1
- Mate:95: 7804K117_Stainless Steel Ball Bearing_MIR:1 ↔ 91290A306_Black-Oxide Alloy Steel Socket Head Screw_MIR:1
- Insert:94: 7804K117_Stainless Steel Ball Bearing_MIR:1 ↔ PivotWasher_MIR:1
- Insert:95: 91290A306_Black-Oxide Alloy Steel Socket Head Screw_MIR:1 ↔ PivotWasher_MIR:1
- Insert:96: CarriagePivotMount_MIR:1 ↔ 90591A255_Zinc-Plated Steel Hex Nut_MIR:1
- Angle:6 (0 deg): ScissorArmV2_MIR:1 ↔ ScissorArmV2Inner_MIR:1
- Mate:96: ScissorArmV2_MIR:1 ↔ ScissorArmV2Inner_MIR:1
- Insert:98: ScissorArmV2_MIR:1 ↔ 7804K117_Stainless Steel Ball Bearing_MIR:3
- Insert:99: ScissorArmV2_MIR:1 ↔ 6656K108_Steel Ball Bearing_MIR:1
- Insert:100: 6656K108_Steel Ball Bearing_MIR:1 ↔ 6656K108_Steel Ball Bearing_MIR:2
- Insert:101: 7804K117_Stainless Steel Ball Bearing_MIR:3 ↔ PivotWasher_MIR:2
- Insert:102: PivotWasher_MIR:2 ↔ 91290A168_Black-Oxide Alloy Steel Socket Head Screw_MIR:1
- Mate:97: ScissorArmV2Inner_MIR:1 ↔ 90591A255_Zinc-Plated Steel Hex Nut_MIR:2
- Insert:103: ScissorArmV2Inner_MIR:1 ↔ 90591A255_Zinc-Plated Steel Hex Nut_MIR:2
- Insert:104: ScissorArmV2_MIR:1 ↔ ThrustBearing_MIR:1
- Insert:105: ScissorArmV2Inner_MIR:1 ↔ ThrustBearing_MIR:2
- Insert:106: CarriagePivotMount_MIR:1 ↔ ThrustBearing_MIR:2
- Insert:107: ScissorArmV2_MIR:1 ↔ 7804K117_Stainless Steel Ball Bearing_MIR:4
- Insert:108: 7804K117_Stainless Steel Ball Bearing_MIR:4 ↔ PivotWasher_MIR:3
- Insert:109: ScissorArmV2_MIR:1 ↔ ThrustBearing_MIR:3
- Mate:99: MGN9-C v2_MIR:1 ↔ UpperCarriagePivotMount_MIR:1
- Mate:100: ThrustBearing_MIR:3 ↔ UpperCarriagePivotMount_MIR:1
- Mate:101: ThrustBearing_MIR:3 ↔ UpperCarriagePivotMount_MIR:1
- Insert:116: PivotWasher_MIR:3 ↔ 91290A306_Black-Oxide Alloy Steel Socket Head Screw_MIR:2
- Mate:106: UpperCarriagePivotMount_MIR:1 ↔ 90591A255_Zinc-Plated Steel Hex Nut_MIR:3
- Insert:117: UpperCarriagePivotMount_MIR:1 ↔ 90591A255_Zinc-Plated Steel Hex Nut_MIR:3
- Angle:8 (0 deg): BottomSideMountRight:1 ↔ MGNRail250mm:3
- Mate:111: MGN9-H:3 ↔ MGNRail250mm:3
- Mate:112: MGN9-H:6 ↔ MGNRail250mm:4
- Flush:30 (5.5 mm): MGN9-H:6 ↔ MGNRail250mm:4
- Insert:123: MGN9-H:6 ↔ XGantryMount:1
- Mate:116: MGN9-H:6 ↔ XGantryMount:1
- Insert:124: MGNRail250mm:3 ↔ XGantryMount:1
- Flush:33 (-5.5 mm): MGN9-H:3 ↔ MGNRail250mm:3
- Mate:117: MGNRail250mm:3 ↔ XGantryMount:1
- Mate:122: MGN9-C v2_MIR:1 ↔ MGNRail250mm:6
- Flush:35 (5.5 mm): MGN9-C v2_MIR:1 ↔ MGNRail250mm:6
- Insert:132: GantryRailMount_MIR:1 ↔ MGNRail250mm:6
- Insert:133: GantryRailMount_MIR:1 ↔ MGNRail250mm:6
- [Mate]: MGN9-H:7 ↔ MGNRail250mm:7
- [Flush] (5.5 mm): MGN9-H:7 ↔ MGNRail250mm:7
- Insert:134: GantryRailMount_MIR:1 ↔ MGNRail250mm:7
- Insert:135: GantryRailMount_MIR:1 ↔ MGNRail250mm:7
- Insert:137: ZBridgePlate:1 ↔ CarriagePivotMount_MIR:1
- Insert:138: XGantryMount:1 ↔ 90729A168_Passivated 316 :4
- Insert:139: XGantryMount:1 ↔ 90729A168_Passivated 316 :3
- Insert:140: XGantryMount:1 ↔ 90729A168_Passivated 316 :1
- Insert:141: XGantryMount:1 ↔ 90729A168_Passivated 316 :2
- Mate:126: XGantryMount:1 ↔ BearingU604:3
- Insert:142: XGantryMount:1 ↔ BearingU604:3
- Insert:143: BearingU604:3 ↔ 91290A306_Black-Oxide Alloy Steel Socket Head Screw:4
- Insert:145: XGantryMount:1 ↔ BearingU604:2
- Insert:146: BearingU604:2 ↔ 91290A306_Black-Oxide Alloy Steel Socket Head Screw:5
- Insert:147: BearingU604:1 ↔ 91290A306_Black-Oxide Alloy Steel Socket Head Screw:6
- Insert:152: MGNRail250mm:4 ↔ ElevatorPlate:1
- Mate:128: MGNRail250mm:4 ↔ ElevatorPlate:1
- Mate:129: ElevatorPlate:1 ↔ 42SHD0034-20B:4
- Angle:10 (0 deg): ElevatorPlate:1 ↔ 42SHD0034-20B:4
- Mate:131: XGantryMount:1 ↔ ElevatorPlate:1
- Mate:132: 42SHD0034-20B:1 ↔ ElevatorPlate_MIR:1
- Flush:39: 42SHD0034-20B:1 ↔ ElevatorPlate_MIR:1
- Flush:40: ElevatorPlate:1 ↔ ElevatorPlate_MIR:1
- Flush:41: ElevatorPlate:1 ↔ ElevatorPlate_MIR:1
- Insert:153: GantryRailMount_MIR:1 ↔ BearingU604:6
- Insert:154: MGN9-H:7 ↔ XGantryMount_MIR:1
- Mate:135: MGN9-H:7 ↔ XGantryMount_MIR:1
- Flush:42: XGantryMount:1 ↔ XGantryMount_MIR:1
- Insert:155: BearingU604:5 ↔ XGantryMount_MIR:1
- Insert:156: BearingU604:4 ↔ XGantryMount_MIR:1
- Insert:157: BearingU604:6 ↔ 91290A306_Black-Oxide Alloy Steel Socket Head Screw:7
- Insert:158: BearingU604:4 ↔ 91290A306_Black-Oxide Alloy Steel Socket Head Screw:8
- Insert:159: BearingU604:5 ↔ 91290A306_Black-Oxide Alloy Steel Socket Head Screw:9
- Insert:160: XGantryMount_MIR:1 ↔ 90729A168_Passivated 316 :12
- Insert:161: XGantryMount_MIR:1 ↔ 90729A168_Passivated 316 :11
- Insert:162: XGantryMount_MIR:1 ↔ 90729A168_Passivated 316 :10
- Insert:163: XGantryMount_MIR:1 ↔ 90729A168_Passivated 316 :9
- Insert:165: 92981A207_Alloy Steel Shoulder Screws:4 ↔ 7804K117_Stainless Steel Ball Bearing:8
- Mate:136: ElevatorPlate:1 ↔ ElevatorShoulderBoltMount:1
- Insert:176: 92981A207_Alloy Steel Shoulder Screws:5 ↔ 7804K117_Stainless Steel Ball Bearing_MIR:5
- Insert:182: ElevatorPlate_MIR:1 ↔ ElevatorShoulderBoltMount_MIR:1
- Mate:138: BottomSideMountRight:1 ↔ MGNRail250mm:8
- Mate:139: BottomSlideMount:1 ↔ MGNRail250mm:9
- Mate:140: BottomSlideMount:1 ↔ MGNRail250mm:9
- Flush:43: BottomSlideMount:1 ↔ MGNRail250mm:9
- Mate:141: BottomSideMountRight:1 ↔ MGNRail250mm:8
- Insert:183: XGantryMount:1 ↔ 91290A306_Black-Oxide Alloy Steel Socket Head Screw:21
- Insert:184: XGantryMount:1 ↔ 91290A306_Black-Oxide Alloy Steel Socket Head Screw:20
- Mate:142: 42SHD0034-20B:4 ↔ Pulley:1
- Mate:143: 42SHD0034-20B:1 ↔ Pulley:2
- Insert:187: BearingU604:12 ↔ Tensioner:1
- Flush:45: 42SHD0034-20B:4 ↔ Pulley:1
- Mate:147: ElevatorPlate:1 ↔ 42SHD0034-20B:4
- Mate:148: 42SHD0034-20B:1 ↔ ElevatorPlate_MIR:1
- Flush:46: 42SHD0034-20B:1 ↔ Pulley:2
- Mate:149: BoundingBox:1 ↔ ElectronicsBase:1
- Mate:152: Pololu Stepper with 300mm LeadScrew:1 ↔ LeadScrewArch:1
- Mate:153: BottomSideMountRight:1 ↔ LeadScrewArch:1
- Mate:154: ZMotorMount:1 ↔ LeadScrewArch:1
- Insert:194: LeadScrewArch:1 ↔ 7804K117_Stainless Steel Ball Bearing:9
- Mate:155: Zeee6S22Ah:1 ↔ LeadScrewArch:1
- Flush:47: BoundingBox:1 ↔ ElectronicsBase:1
- Mate:156: ElectronicsBase:1 ↔ FrontPanel:2
- Flush:49: ElectronicsBase:1 ↔ FrontPanel:2
- Insert:197: FrontPanel:2 ↔ 7804K117_Stainless Steel Ball Bearing:10
- Insert:198: knob:1 ↔ 7804K117_Stainless Steel Ball Bearing:10
- Angle:11 (0 deg): FrontPanel:2 ↔ BTT Mini 12864 V1.0:1
- Insert:199: FrontPanel:2 ↔ BTT Mini 12864 V1.0:1
- Insert:200: FrontPanel:2 ↔ BTT Mini 12864 V1.0:1
- Insert:201: FrontPanel:2 ↔ 90729A168_Passivated 316 :13
- Insert:202: FrontPanel:2 ↔ 90729A168_Passivated 316 :14
- Insert:203: ElectronicsBase:1 ↔ 90729A168_Passivated 316 :15
- Insert:206: ElectronicsBase:1 ↔ 90729A168_Passivated 316 :16
- Insert:207: BottomSlideMount:1 ↔ BottomSlideMountExtension:1
- Insert:208: BottomSlideMount:1 ↔ BottomSlideMountExtension:1
- Insert:210: ElectronicsBase:1 ↔ 90729A168_Passivated 316 :17
- Insert:211: BottomSlideMountExtension_MIR:1 ↔ RightTruss:1
- Insert:212: BottomSlideMountExtension:1 ↔ LeftTruss:1
- Insert:213: BottomSlideMount:1 ↔ LeftTruss:1
- Insert:214: ElectronicsBase:1 ↔ 90729A168_Passivated 316 :19
- Insert:215: ElectronicsBase:1 ↔ 90729A168_Passivated 316 :20
- Insert:216: ElevatorPlate:1 ↔ RoutingPlateV2:1
- Insert:217: ElevatorPlate:1 ↔ RoutingPlateV2:1
- Mate:159 (0.1 mm): Tensioner:1 ↔ RoutingPlateV2:1
- Insert:218: BearingU604:10 ↔ RoutingPlateV2:1
- Insert:219: BearingU604:10 ↔ 91290A306_Black-Oxide Alloy Steel Socket Head Screw:22
- Insert:220: Tensioner:1 ↔ 91290A306_Black-Oxide Alloy Steel Socket Head Screw:23
- Insert:221: RoutingPlateV2:1 ↔ BearingU604:18
- Insert:222: BearingU604:18 ↔ 91290A306_Black-Oxide Alloy Steel Socket Head Screw:24
- Insert:223: ElevatorPlate_MIR:1 ↔ RoutingPlateV2Right:1
- Mate:163: ElevatorShoulderBoltMount_MIR:1 ↔ RoutingPlateV2Right:1
- Insert:225: RoutingPlateV2Right:1 ↔ BearingU604:19
- [Insert]: BearingU604:21 ↔ Tensioner:2
- [Insert]: Tensioner:2 ↔ 91290A306_Black-Oxide Alloy Steel Socket Head Screw:25
- Mate:164 (0.1 mm): RoutingPlateV2Right:1 ↔ Tensioner:2
- Insert:228: RoutingPlateV2Right:1 ↔ BearingU604:22
- Insert:229: BearingU604:17 ↔ RoutingPlateV2Right:1
- Insert:230: BearingU604:22 ↔ 91290A306_Black-Oxide Alloy Steel Socket Head Screw:26
- Insert:231: BearingU604:17 ↔ 91290A306_Black-Oxide Alloy Steel Socket Head Screw:27
- Insert:232: BearingU604:19 ↔ 91290A306_Black-Oxide Alloy Steel Socket Head Screw:28
- Insert:233: Raspberry PI Zero W:1 ↔ BottomSlideMountExtension:1
- Mate:166: Raspberry PI Zero W:1 ↔ BottomSlideMountExtension:1
- Mate:167: Zeee6S22Ah:1 ↔ BottomSlideMount:1
- Insert:234 (3 mm): BTT E3 SKR MINI V3.0:1 ↔ BottomSlideMountExtension_MIR:1
- Mate:168: BottomSideMountRight:1 ↔ BottomSlideMountExtension_MIR:1
- Mate:169: BTT E3 SKR MINI V3.0:1 ↔ BottomSideMountRight:1
- Insert:241: ThrustBearing_MIR:1 ↔ ShoulderBoltMountV2_MIR:1
- Mate:170: BottomSlideMount:1 ↔ ShoulderBoltMountV2_MIR:1
- Mate:171: BottomSlideMount:1 ↔ ShoulderBoltMountV2_MIR:1
- Flush:50: BottomSlideMount:1 ↔ ShoulderBoltMountV2_MIR:1
- Insert:243: FrontPanel:2 ↔ 90729A168_Passivated 316 :28
- Insert:244: FrontPanel:2 ↔ 90729A168_Passivated 316 :29
- Insert:245: FrontPanel:2 ↔ 90729A168_Passivated 316 :30
- Insert:246: FrontPanel:2 ↔ 90729A168_Passivated 316 :31
- Insert:247: MGNRail250mm:7 ↔ 91290A110_Black-Oxide Alloy Steel Socket Head Screw_MIR:5
- Mate:172: BottomSideMountRight:1 ↔ BottomSlideMountExtension_MIR:1
- Insert:248: RoutingPlateV2:1 ↔ 91290A306_Black-Oxide Alloy Steel Socket Head Screw:32
- Insert:249: RoutingPlateV2:1 ↔ 91290A306_Black-Oxide Alloy Steel Socket Head Screw:29
- Insert:250: RoutingPlateV2:1 ↔ 91290A306_Black-Oxide Alloy Steel Socket Head Screw:31
- Insert:251: RoutingPlateV2:1 ↔ 91290A306_Black-Oxide Alloy Steel Socket Head Screw:30
- Insert:252: RoutingPlateV2Right:1 ↔ 91290A306_Black-Oxide Alloy Steel Socket Head Screw:35
- Insert:253: RoutingPlateV2Right:1 ↔ 91290A306_Black-Oxide Alloy Steel Socket Head Screw:36
- Insert:254: RoutingPlateV2Right:1 ↔ 91290A306_Black-Oxide Alloy Steel Socket Head Screw:34
- Insert:255: RoutingPlateV2Right:1 ↔ 91290A306_Black-Oxide Alloy Steel Socket Head Screw:33
- Insert:256: RoutingPlateV2Right:1 ↔ 91290A110_Black-Oxide Alloy Steel Socket Head Screw_MIR:32
- Insert:257: RoutingPlateV2:1 ↔ 91290A110_Black-Oxide Alloy Steel Socket Head Screw_MIR:31
- Insert:258: ElevatorPlate:1 ↔ 91290A110_Black-Oxide Alloy Steel Socket Head Screw_MIR:33
- Insert:259: ElevatorPlate_MIR:1 ↔ 91290A110_Black-Oxide Alloy Steel Socket Head Screw_MIR:37
- Insert:260: MGNRail250mm:3 ↔ 91290A110_Black-Oxide Alloy Steel Socket Head Screw_MIR:41
- Insert:261: BottomSlideMount:1 ↔ 91290A110_Black-Oxide Alloy Steel Socket Head Screw_MIR:54
- Insert:263: LeadScrewArch:1 ↔ 91290A110_Black-Oxide Alloy Steel Socket Head Screw_MIR:60
- Insert:264: Raspberry PI Zero W:1 ↔ 91290A110_Black-Oxide Alloy Steel Socket Head Screw_MIR:61
- Insert:265: Raspberry PI Zero W:1 ↔ 91290A110_Black-Oxide Alloy Steel Socket Head Screw_MIR:62
- Insert:266: ZMotorMount:1 ↔ 91290A306_Black-Oxide Alloy Steel Socket Head Screw:38
- Insert:267: ZMotorMount:1 ↔ 91290A306_Black-Oxide Alloy Steel Socket Head Screw:39
- Insert:268: ZMotorMount:1 ↔ 91290A306_Black-Oxide Alloy Steel Socket Head Screw:40
- Insert:269: ZMotorMount:1 ↔ 91290A306_Black-Oxide Alloy Steel Socket Head Screw:41
- Insert:270: ZMotorMount:1 ↔ 91290A306_Black-Oxide Alloy Steel Socket Head Screw:42
- Insert:271: ZMotorMount:1 ↔ 91290A306_Black-Oxide Alloy Steel Socket Head Screw:43
- Insert:272: ZMotorMount:1 ↔ 91290A306_Black-Oxide Alloy Steel Socket Head Screw:44
- Insert:273: ShoulderBoltMountV2:1 ↔ 91290A306_Black-Oxide Alloy Steel Socket Head Screw:46
- Insert:274: ShoulderBoltMountV2:1 ↔ 91290A306_Black-Oxide Alloy Steel Socket Head Screw:47
- Insert:275: ShoulderBoltMountV2:1 ↔ 91290A306_Black-Oxide Alloy Steel Socket Head Screw:48
- Insert:276: ShoulderBoltMountV2:1 ↔ 91290A306_Black-Oxide Alloy Steel Socket Head Screw:49
- Insert:277: ShoulderBoltMountV2:1 ↔ 91290A306_Black-Oxide Alloy Steel Socket Head Screw:50
- Insert:278: ShoulderBoltMountV2_MIR:1 ↔ 91290A306_Black-Oxide Alloy Steel Socket Head Screw:51
- Insert:279: ShoulderBoltMountV2_MIR:1 ↔ 91290A306_Black-Oxide Alloy Steel Socket Head Screw:52
- Insert:280: ShoulderBoltMountV2_MIR:1 ↔ 91290A306_Black-Oxide Alloy Steel Socket Head Screw:53
- Insert:281: ShoulderBoltMountV2_MIR:1 ↔ 91290A306_Black-Oxide Alloy Steel Socket Head Screw:54
- Insert:282: ShoulderBoltMountV2_MIR:1 ↔ 91290A306_Black-Oxide Alloy Steel Socket Head Screw:55
- Insert:283: BottomSideMountRight:1 ↔ 91290A306_Black-Oxide Alloy Steel Socket Head Screw:56
- Insert:284: BottomSlideMountExtension_MIR:1 ↔ 91290A306_Black-Oxide Alloy Steel Socket Head Screw:60
- Insert:285: MGNRail250mm:9 ↔ 91290A110_Black-Oxide Alloy Steel Socket Head Screw_MIR:63
- Insert:287: MGNRail250mm:6 ↔ 91290A110_Black-Oxide Alloy Steel Socket Head Screw_MIR:102
- Insert:288: ShoulderBoltMountV2_MIR:1 ↔ 91290A110_Black-Oxide Alloy Steel Socket Head Screw_MIR:115
- Insert:289: ShoulderBoltMountV2_MIR:1 ↔ 91290A110_Black-Oxide Alloy Steel Socket Head Screw_MIR:116
- Insert:290: ShoulderBoltMountV2:1 ↔ 91290A110_Black-Oxide Alloy Steel Socket Head Screw_MIR:117
- Insert:291: ShoulderBoltMountV2:1 ↔ 91290A110_Black-Oxide Alloy Steel Socket Head Screw_MIR:118
- Insert:292: UpperCarriagePivotMount:1 ↔ 92095A181_NO THREAD:4
- Insert:293: UpperCarriagePivotMount:1 ↔ 92095A181_NO THREAD:3
- Insert:294: UpperCarriagePivotMount:1 ↔ 92095A181_NO THREAD:2
- Insert:295: UpperCarriagePivotMount:1 ↔ 92095A181_NO THREAD:1
- Insert:296: UpperCarriagePivotMount_MIR:1 ↔ 92095A181_NO THREAD:5
- Insert:297: UpperCarriagePivotMount_MIR:1 ↔ 92095A181_NO THREAD:6
- Insert:298: UpperCarriagePivotMount_MIR:1 ↔ 92095A181_NO THREAD:7
- Insert:299: UpperCarriagePivotMount_MIR:1 ↔ 92095A181_NO THREAD:8
- Insert:300: ZBridgePlate:1 ↔ 92095A181_NO THREAD:9
- Insert:301: ZBridgePlate:1 ↔ 92095A181_NO THREAD:11
- Insert:302: ZBridgePlate:1 ↔ 92095A181_NO THREAD:10
- Insert:303: ZMotorMount:1 ↔ 91290A110_Black-Oxide Alloy Steel Socket Head Screw_MIR:119
- Insert:306: LeadScrewArch:1 ↔ 91290A110_Black-Oxide Alloy Steel Socket Head Screw_MIR:125
- Mate:173: 90729A168_Passivated 316 :7 ↔ MockCable:1
- Mate:174 (2.5 mm): XGantryMount:1 ↔ MockCable:1